# Autodesk Inventor assembly: sparFullFlat_SA
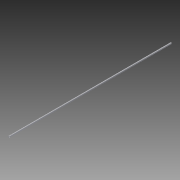
[picture p0: Inventor's stored thumbnail of the model, 180x180]
Saved by Autodesk Inventor 2014 (Build 180170000, 170)
## iProperties
Created: 2015-03-31
Part Number: sparFullFlat_SA
Document SubType Name: Assembly
Designer: ddeboer
Author: ddeboer
## Documents named in this file (4)
- C:\Users\ddeboer\Desktop\hera-cad\surface\sparFullFlat_SA.iam
- C:\Users\ddeboer\Desktop\hera-cad\surface\pvcSection_63mm.ipt
- C:\Users\ddeboer\Desktop\hera-cad\smallParts\coupler_63mm.ipt
- C:\Users\ddeboer\Desktop\hera-cad\surface\pvcSection_63mm_cut4full.ipt
## Components (3 placed, 3 different names)
1. pvcSection_63mm:1 — Insert:1
2. coupler_63mm:1 — Insert:1, Insert:2
3. pvcSection_63mm_cut4full:1 — Insert:2
## Relationships (2: Insert 2)
- Insert:1 (-29 mm): pvcSection_63mm:1 ↔ coupler_63mm:1
- Insert:2 (-29 mm): coupler_63mm:1 ↔ pvcSection_63mm_cut4full:1
